# Autodesk Inventor assembly: assy_three_way_intersection_left_open
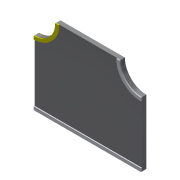
[picture p0: Inventor's stored thumbnail of the model, 180x180]
Saved by Autodesk Inventor 2018 (Build 220112000, 112)
## iProperties
Created: 2017-11-13
Part Number: assy_three_way_intersection_left_open
Document SubType Name: Assembly
Designer: Platform
Author: Platform
## Documents named in this file (4)
- C:\Users\Platform\Desktop\autorace_track\track_model\autorace_rbizchallenge2017\assembled\assy_three_way_intersection_left_open.iam
- C:\Users\Platform\Desktop\autorace_track\track_model\autorace_rbizchallenge2017\parts\ipt\upper_plate_crossway v1.ipt
- C:\Users\Platform\Desktop\autorace_track\track_model\autorace_rbizchallenge2017\parts\ipt\straight_line.ipt
- C:\Users\Platform\Desktop\autorace_track\track_model\autorace_rbizchallenge2017\parts\ipt\curved_line_sml.ipt
## Components (4 placed, 3 different names)
1. upper_plate_crossway v1:1
2. straight_line:1
3. curved_line_sml:1
4. curved_line_sml:2
## Relationships (4: Mate 4)
- [Mate]: upper_plate_crossway v1:1 ↔ straight_line:1
- [Mate]: upper_plate_crossway v1:1 ↔ straight_line:1
- [Mate]: upper_plate_crossway v1:1 ↔ curved_line_sml:1
- [Mate]: upper_plate_crossway v1:1 ↔ curved_line_sml:2
